# Autodesk Inventor assembly: ASY MSC 201 BACK
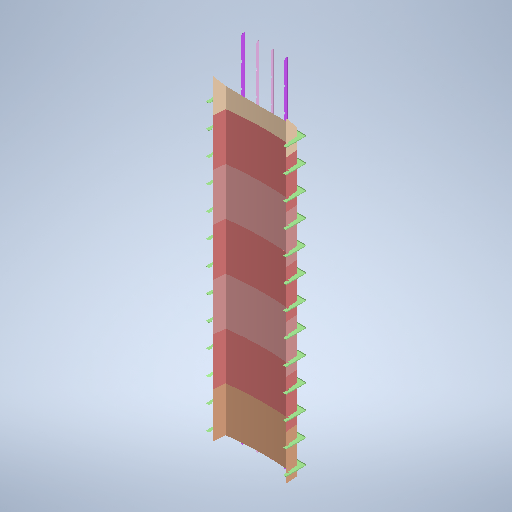
[picture p0: Inventor's stored thumbnail of the model, 512x512]
Saved by Autodesk Inventor 2025 (Build 290162010, 162A)
## iProperties
Created: 2024-07-19
Part Number: ASY MSC 201 BACK
Document SubType Name: Assembly
Designer: pokla
Author: pokla
## Documents named in this file (8)
- C:\Users\user\YandexDisk\домашниий пк\Inventor\Manturovo\Manturovo_Se-clar\ASY MSC 201 BACK.iam
- C:\Users\user\YandexDisk\домашниий пк\Inventor\Manturovo\Manturovo_Se-clar\MSC 033 sheet back basic.ipt
- C:\Users\user\YandexDisk\домашниий пк\Inventor\Manturovo\Manturovo_Se-clar\MSC 051 rib back.ipt
- C:\Users\user\YandexDisk\домашниий пк\Inventor\Manturovo\Manturovo_Se-clar\MSC 032 sheet magic back-lowerback.ipt
- C:\Users\user\YandexDisk\домашниий пк\Inventor\Manturovo\Manturovo_Se-clar\MSC 034 sheet back-neck.ipt
- C:\Users\user\YandexDisk\домашниий пк\Inventor\Manturovo\Manturovo_Se-clar\MSC 061 stringer back ^.ipt
- C:\Users\user\YandexDisk\домашниий пк\Inventor\Manturovo\Manturovo_Se-clar\MSC 062 stringer back ^^.ipt
- C:\Users\user\YandexDisk\домашниий пк\Inventor\Manturovo\Manturovo_Se-clar\MSC 0331 sheet back mould.ipt
## Components (66 placed, 10 different names)
1. MSC 033 sheet back basic.ipt:1
2. MSC 051 rib back.ipt:6
3. MSC 033 sheet back basic.ipt:2
4. MSC 033 sheet back basic.ipt:3 — Mate:1, Flush:2, Tangent:2, Mate:2
5. MSC 051 rib back.ipt:1
6. MSC 032 sheet magic back-lowerback.ipt:1 — Mate:2, Flush:3
7. MSC 033 sheet back basic.ipt:4
8. MSC 033 sheet back basic.ipt:5
9. MSC 034 sheet back-neck.ipt:1
10. MSC 061 stringer back ^.ipt:1
11. MSC 061 stringer back ^.ipt:2
12. MSC 062 stringer back ^^.ipt:2
13. MSC 062 stringer back ^^.ipt:1
14. MSC 051 rib back.ipt:2
15. MSC 051 rib back.ipt:3
16. MSC 051 rib back.ipt:4
17. MSC 051 rib back.ipt:5 — Flush:3
18. MSC 051 rib back.ipt:8 — Rigid:41
19. MSC 051 rib back.ipt:7
20. MSC 061 stringer back ^.ipt:4 — Rigid:61
21. MSC 061 stringer back ^.ipt:3 — Rigid:62
22. MSC 062 stringer back ^^.ipt:4 — Rigid:60
23. MSC 062 stringer back ^^.ipt:3 — Rigid:63
24. MSC 0331 sheet back mould:1 — Mate:1, Flush:2, Tangent:2, Rigid:22, Rigid:23
25. MSC 0331 sheet back mould:2 — Rigid:22, Rigid:25
26. MSC 0331 sheet back mould:3 — Rigid:23, Rigid:24
27. MSC 0331 sheet back mould:4 — Rigid:24
28. MSC 0331 sheet back mould:5 — Rigid:25, Rigid:27
29. MSC 0331 sheet back mould:6 — Rigid:27
30. MSC 0331 sheet back mould:7 — Rigid:31
31. MSC 0331 sheet back mould:8 — Rigid:31
32. MSC 0331 sheet back mould:9
33. MSC 0331 sheet back mould:10
34. MSC 0331 sheet back mould:11 — Rigid:33
35. MSC 0331 sheet back mould:12 — Rigid:33
36. MSC 0331 sheet back mould:13
37. MSC 051 rib back:10
38. MSC 051 rib back:11
39. MSC 051 rib back:12
40. MSC 051 rib back:13
41. MSC 051 rib back:14 — Rigid:41
42. MSC 051 rib back:15
43. MSC 051 rib back:16 — Rigid:51
44. MSC 051 rib back:17
45. MSC 051 rib back:18 — Rigid:51
46. MSC 051 rib back:19
47. MSC 051 rib back:20
48. MSC 051 rib back:21
49. MSC 051 rib back:22
50. MSC 051 rib back:23
51. MSC 051 rib back:24
52. MSC 051 rib back:25
53. MSC 051 rib back:26
54. MSC 051 rib back:27
55. МОО 051 стрингер спина 1:6 — Rigid:62
56. МОО 051 стрингер спина 1:7 — Rigid:61
57. МОО 052 стрингер спина 2:6 — Rigid:63
58. МОО 052 стрингер спина 2:7 — Rigid:60
59. МОО 051 стрингер спина 1:8 — Rigid:57
60. МОО 051 стрингер спина 1:9 — Rigid:58
61. МОО 052 стрингер спина 2:8 — Rigid:56
62. МОО 052 стрингер спина 2:9 — Rigid:59
63. МОО 052 стрингер спина 2:10 — Rigid:56
64. МОО 051 стрингер спина 1:10 — Rigid:57
65. МОО 051 стрингер спина 1:11 — Rigid:58
66. МОО 052 стрингер спина 2:11 — Rigid:59
## Relationships (70: WeldJoint 63, Flush 3, Tangent 2, Mate 2)
- [WeldJoint]: MSC 033 sheet back basic.ipt:1 ↔ MSC 033 sheet back basic.ipt:2
- [WeldJoint]: MSC 033 sheet back basic.ipt:1 ↔ MSC 033 sheet back basic.ipt:3
- [Tangent]: MSC 051 rib back.ipt:6 ↔ MSC 033 sheet back basic.ipt:2
- [WeldJoint] (-50 mm): MSC 051 rib back.ipt:6 ↔ MSC 051 rib back.ipt:1
- [WeldJoint]: MSC 033 sheet back basic.ipt:3 ↔ MSC 032 sheet magic back-lowerback.ipt:1
- [WeldJoint]: MSC 033 sheet back basic.ipt:2 ↔ MSC 033 sheet back basic.ipt:4
- [WeldJoint]: MSC 033 sheet back basic.ipt:4 ↔ MSC 033 sheet back basic.ipt:5
- [WeldJoint]: MSC 033 sheet back basic.ipt:5 ↔ MSC 034 sheet back-neck.ipt:1
- [Flush] (-250 mm): MSC 051 rib back.ipt:6 ↔ MSC 033 sheet back basic.ipt:3
- [WeldJoint] (2 mm): MSC 051 rib back.ipt:6 ↔ MSC 061 stringer back ^.ipt:1
- [WeldJoint] (2 mm): MSC 051 rib back.ipt:1 ↔ MSC 061 stringer back ^.ipt:2
- [WeldJoint] (2 mm): MSC 051 rib back.ipt:6 ↔ MSC 062 stringer back ^^.ipt:2
- [WeldJoint] (2 mm): MSC 051 rib back.ipt:1 ↔ MSC 062 stringer back ^^.ipt:1
- [WeldJoint] (50 mm): MSC 051 rib back.ipt:2 ↔ MSC 051 rib back.ipt:3
- [WeldJoint] (50 mm): MSC 051 rib back.ipt:4 ↔ MSC 051 rib back.ipt:5
- [WeldJoint] (-500 mm): MSC 051 rib back.ipt:6 ↔ MSC 051 rib back.ipt:2
- [WeldJoint] (-500 mm): MSC 051 rib back.ipt:2 ↔ MSC 051 rib back.ipt:4
- [WeldJoint] (-50 mm): MSC 051 rib back.ipt:8 ↔ MSC 051 rib back.ipt:7
- [WeldJoint] (-500 mm): MSC 051 rib back.ipt:1 ↔ MSC 051 rib back.ipt:7
- [WeldJoint]: MSC 061 stringer back ^.ipt:1 ↔ MSC 061 stringer back ^.ipt:3
- [WeldJoint]: MSC 061 stringer back ^.ipt:2 ↔ MSC 061 stringer back ^.ipt:4
- [WeldJoint]: MSC 062 stringer back ^^.ipt:2 ↔ MSC 062 stringer back ^^.ipt:3
- [WeldJoint]: MSC 062 stringer back ^^.ipt:1 ↔ MSC 062 stringer back ^^.ipt:4
- Mate:1: MSC 033 sheet back basic.ipt:3 ↔ MSC 0331 sheet back mould:1
- Flush:2 (248.5 mm): MSC 033 sheet back basic.ipt:3 ↔ MSC 0331 sheet back mould:1
- Tangent:2: MSC 033 sheet back basic.ipt:3 ↔ MSC 0331 sheet back mould:1
- Rigid:22 [WeldJoint] (497 mm): MSC 0331 sheet back mould:1 ↔ MSC 0331 sheet back mould:2
- Rigid:23 [WeldJoint] (497 mm): MSC 0331 sheet back mould:1 ↔ MSC 0331 sheet back mould:3
- Rigid:24 [WeldJoint] (497 mm): MSC 0331 sheet back mould:3 ↔ MSC 0331 sheet back mould:4
- Rigid:25 [WeldJoint] (497 mm): MSC 0331 sheet back mould:2 ↔ MSC 0331 sheet back mould:5
- [WeldJoint] (497 mm): MSC 0331 sheet back mould:6 ↔ MSC 0331 sheet back mould:7
- Rigid:27 [WeldJoint] (497 mm): MSC 0331 sheet back mould:5 ↔ MSC 0331 sheet back mould:6
- [WeldJoint] (497 mm): MSC 0331 sheet back mould:8 ↔ MSC 0331 sheet back mould:9
- [WeldJoint] (497 mm): MSC 0331 sheet back mould:10 ↔ MSC 0331 sheet back mould:11
- [WeldJoint] (497 mm): MSC 0331 sheet back mould:9 ↔ MSC 0331 sheet back mould:10
- Rigid:31 [WeldJoint] (497 mm): MSC 0331 sheet back mould:7 ↔ MSC 0331 sheet back mould:8
- [WeldJoint] (497 mm): MSC 0331 sheet back mould:12 ↔ MSC 0331 sheet back mould:13
- Rigid:33 [WeldJoint] (497 mm): MSC 0331 sheet back mould:11 ↔ MSC 0331 sheet back mould:12
- Mate:2: MSC 033 sheet back basic.ipt:3 ↔ MSC 032 sheet magic back-lowerback.ipt:1
- Flush:3: MSC 032 sheet magic back-lowerback.ipt:1 ↔ MSC 051 rib back.ipt:5
- [WeldJoint] (-50 mm): MSC 051 rib back:10 ↔ MSC 051 rib back:11
- [WeldJoint] (50 mm): MSC 051 rib back:12 ↔ MSC 051 rib back:13
- [WeldJoint] (50 mm): MSC 051 rib back:14 ↔ MSC 051 rib back:15
- [WeldJoint] (-500 mm): MSC 051 rib back:10 ↔ MSC 051 rib back:12
- [WeldJoint] (-500 mm): MSC 051 rib back:12 ↔ MSC 051 rib back:14
- [WeldJoint] (-50 mm): MSC 051 rib back:16 ↔ MSC 051 rib back:17
- [WeldJoint] (-500 mm): MSC 051 rib back:11 ↔ MSC 051 rib back:17
- Rigid:41 [WeldJoint] (-500 mm): MSC 051 rib back.ipt:8 ↔ MSC 051 rib back:14
- [WeldJoint] (-50 mm): MSC 051 rib back:18 ↔ MSC 051 rib back:19
- [WeldJoint] (-50 mm): MSC 051 rib back:20 ↔ MSC 051 rib back:21
- [WeldJoint] (50 mm): MSC 051 rib back:22 ↔ MSC 051 rib back:23
- [WeldJoint] (50 mm): MSC 051 rib back:24 ↔ MSC 051 rib back:25
- [WeldJoint] (-500 mm): MSC 051 rib back:20 ↔ MSC 051 rib back:22
- [WeldJoint] (-500 mm): MSC 051 rib back:22 ↔ MSC 051 rib back:24
- [WeldJoint] (-50 mm): MSC 051 rib back:26 ↔ MSC 051 rib back:27
- [WeldJoint] (-500 mm): MSC 051 rib back:21 ↔ MSC 051 rib back:27
- [WeldJoint] (-500 mm): MSC 051 rib back:18 ↔ MSC 051 rib back:24
- Rigid:51 [WeldJoint] (-500 mm): MSC 051 rib back:16 ↔ MSC 051 rib back:18
- [WeldJoint]: МОО 051 стрингер спина 1:6 ↔ МОО 051 стрингер спина 1:9
- [WeldJoint]: МОО 051 стрингер спина 1:7 ↔ МОО 051 стрингер спина 1:8
- [WeldJoint]: МОО 052 стрингер спина 2:6 ↔ МОО 052 стрингер спина 2:9
- [WeldJoint]: МОО 052 стрингер спина 2:7 ↔ МОО 052 стрингер спина 2:8
- Rigid:56 [WeldJoint]: МОО 052 стрингер спина 2:8 ↔ МОО 052 стрингер спина 2:10
- Rigid:57 [WeldJoint]: МОО 051 стрингер спина 1:8 ↔ МОО 051 стрингер спина 1:10
- Rigid:58 [WeldJoint]: МОО 051 стрингер спина 1:9 ↔ МОО 051 стрингер спина 1:11
- Rigid:59 [WeldJoint]: МОО 052 стрингер спина 2:9 ↔ МОО 052 стрингер спина 2:11
- Rigid:60 [WeldJoint]: MSC 062 stringer back ^^.ipt:4 ↔ МОО 052 стрингер спина 2:7
- Rigid:61 [WeldJoint]: MSC 061 stringer back ^.ipt:4 ↔ МОО 051 стрингер спина 1:7
- Rigid:62 [WeldJoint]: MSC 061 stringer back ^.ipt:3 ↔ МОО 051 стрингер спина 1:6
- Rigid:63 [WeldJoint]: MSC 062 stringer back ^^.ipt:3 ↔ МОО 052 стрингер спина 2:6
## Named parameters: d390_d128 = -50 mm, d322_d320 = 50 mm, d42_d41 = 497 mm, d44_d41 = 497 mm, d45_d42_d41 = 497 mm, d46_d43 = 497 mm, d48_d45_d42_d41 = 497 mm, d52_d362 = -500 mm, d53_d363 = -500 mm, d54_d390_d128 = -50 mm, d55_d391 = -500 mm, d56_d320 = 50 mm, d57_d322_d320 = 50 mm, d58_d128 = -50 mm, d60_d390_d128 = -50 mm, d61_d52_d362 = -500 mm, d62_d53_d363 = -500 mm, d63_d54_d390_d128 = -50 mm, d64_d55_d391 = -500 mm, d65_d56_d320 = 50 mm, d66_d57_d322_d320 = 50 mm, d67_d58_d128 = -50 mm, d68_d59 = -500 mm, d70_d408 = 0 mm, d71_d409 = 0 mm, d72_d410 = 0 mm, d73_d411 = 0 mm
